# Autodesk Inventor assembly: HexMotorDirectDrive
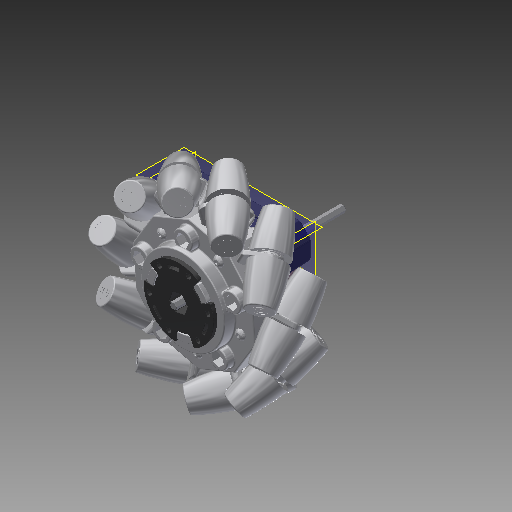
[picture p0: Inventor's stored thumbnail of the model, 512x512]
Saved by Autodesk Inventor 2017 (Build 210142000, 142)
## iProperties
Created: 2017-12-02
Part Number: HexMotorDirectDrive
Document SubType Name: Assembly
Designer: User
Author: User
## Documents named in this file (6)
- C:\Robotics\CAD\2017-18_CAD\Prototypes\HexMotorDirectDrive.iam
- C:\Robotics\CAD\COTSParts\Rev\REV-41-1300.ipt
- C:\Robotics\CAD\COTSParts\Vex\6inchMecanumRight217-2586-STEP\6inchMecanumRight217-2586.20121203.ipt
- C:\Robotics\CAD\COTSParts\Vex\VersaHub.5inchBore217-4009-STEP-20140807\VersaHub.5inchBore217-4009-STEP-20140807.ipt
- C:\Robotics\CAD\COTSParts\Rev\REV-41-1147HexHub.ipt
- C:\Robotics\CAD\COTSParts\Rev\REV-41-1349.ipt
## Components (6 placed, 5 different names)
1. REV-41-1300:1 — Mate:7, Mate:8, Flush:1, Mate:11
2. 6inchMecanumRight217-2586.20121203:1 — Mate:1, Mate:2, Mate:3, Mate:4, Mate:5, Mate:6, Mate:10
3. VersaHub.5inchBore217-4009-STEP-20140807:1 — Mate:1, Mate:2, Mate:3, Mate:9, Mate:14
4. VersaHub.5inchBore217-4009-STEP-20140807:2 — Mate:4, Mate:5, Mate:6, Flush:2
5. REV-41-1147HexHub:2 — Mate:9, Mate:10, Mate:11, Mate:12, Mate:13, Mate:14
6. REV-41-1349:1 — Mate:7, Mate:8, Flush:1, Flush:2, Mate:12, Mate:13
## Relationships (16: Mate 14, Flush 2)
- Mate:1: 6inchMecanumRight217-2586.20121203:1 ↔ VersaHub.5inchBore217-4009-STEP-20140807:1
- Mate:2: 6inchMecanumRight217-2586.20121203:1 ↔ VersaHub.5inchBore217-4009-STEP-20140807:1
- Mate:3: 6inchMecanumRight217-2586.20121203:1 ↔ VersaHub.5inchBore217-4009-STEP-20140807:1
- Mate:4: 6inchMecanumRight217-2586.20121203:1 ↔ VersaHub.5inchBore217-4009-STEP-20140807:2
- Mate:5: 6inchMecanumRight217-2586.20121203:1 ↔ VersaHub.5inchBore217-4009-STEP-20140807:2
- Mate:6: 6inchMecanumRight217-2586.20121203:1 ↔ VersaHub.5inchBore217-4009-STEP-20140807:2
- Mate:7: REV-41-1300:1 ↔ REV-41-1349:1
- Mate:8: REV-41-1300:1 ↔ REV-41-1349:1
- Flush:1 (-39.6748 mm): REV-41-1300:1 ↔ REV-41-1349:1
- Flush:2: VersaHub.5inchBore217-4009-STEP-20140807:2 ↔ REV-41-1349:1
- Mate:9: VersaHub.5inchBore217-4009-STEP-20140807:1 ↔ REV-41-1147HexHub:2
- Mate:10: 6inchMecanumRight217-2586.20121203:1 ↔ REV-41-1147HexHub:2
- Mate:11 (3.81 mm): REV-41-1300:1 ↔ REV-41-1147HexHub:2
- Mate:12: REV-41-1147HexHub:2 ↔ REV-41-1349:1
- Mate:13: REV-41-1147HexHub:2 ↔ REV-41-1349:1
- Mate:14: VersaHub.5inchBore217-4009-STEP-20140807:1 ↔ REV-41-1147HexHub:2
